# Autodesk Inventor assembly: Baugruppe1
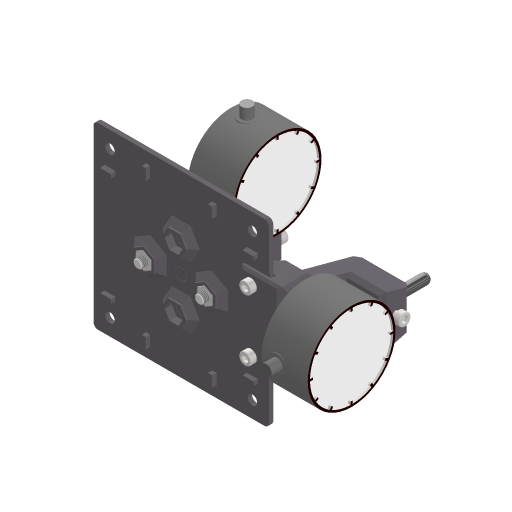
[picture p0: Inventor's stored thumbnail of the model, 512x512]
Saved by Autodesk Inventor 2023.2 (Build 272271000, 271)
## iProperties
Created: 2024-12-10
Part Number: Baugruppe1
Document SubType Name: Assembly
Designer: Nils Bade
Author: Nils Bade
## Documents named in this file (11)
- C:\Users\nilsb\Documents\Inventor\Projektarbeit-Bade\RatRig_modified\ProbeHead\ProbeAntennas\Vermessungsbauteile\MessuhrHalterAssembly.iam
- MessuhrHalterAssembly.iam
- C:\Users\nilsb\Documents\Inventor\Projektarbeit-Bade\RatRig_modified\ProbeHead\ProbeAntennas\Vermessungsbauteile\MessuhrHalter-BasePlate.ipt
- C:\Users\nilsb\Documents\Inventor\Projektarbeit-Bade\RatRig_modified\ProbeHead\ProbeAntennas\Vermessungsbauteile\MessuhrXYKlemme.ipt
- C:\Users\nilsb\Documents\Inventor\Projektarbeit-Bade\RatRig_modified\ProbeHead\ProbeAntennas\Vermessungsbauteile\MessuhrZKlemme.ipt
- C:\Users\nilsb\Documents\Inventor\Projektarbeit-Bade\RatRig_modified\ProbeHead\ProbeAntennas\Vermessungsbauteile\Messuhr-Dummy.ipt
- C:\Users\nilsb\Documents\Inventor\Projektarbeit-Bade\Schrauben\Cap Head Screw M3x12 v2.ipt
- C:\Users\nilsb\Documents\Inventor\Projektarbeit-Bade\Schrauben\Cap Head Screw M3x8 v2.ipt
- C:\Users\nilsb\Documents\Inventor\Projektarbeit-Bade\RatRig_Standards\Hex Nut - M3 v2.ipt
- C:\Users\nilsb\Documents\Inventor\Projektarbeit-Bade\RatRig_Standards\Hex Nut - M4 DIN934.ipt
- C:\Users\nilsb\Documents\Inventor\Projektarbeit-Bade\Schrauben\Cap Head Screw M4x10 - DIN912.ipt
## Components (18 placed, 9 different names)
1. MessuhrHalter-BasePlate:1 — Passend:1, Passend:2, Passend:3, Passend:4, Passend:5, Passend:6, Passend:27, Passend:28, Winkel:5, Winkel:6, Passend:29, Passend:30
2. MessuhrXYKlemme:1 — Passend:1, Passend:2, Passend:6, Tangential:2, Passend:8, Passend:10, Passend:11, Passend:12, Passend:13, Winkel:1, Winkel:2, Passend:17, Passend:18, Passend:31, Passend:32, Passend:33, Passend:34
3. MessuhrZKlemme:1 — Passend:3, Passend:4, Passend:5, Passend:7, Tangential:1, Passend:9, Passend:14, Passend:19, Passend:20, Passend:21, Passend:22, Winkel:3, Winkel:4, Passend:25, Passend:26
4. Messuhr-Dummy:1 — Tangential:2, Passend:8
5. Messuhr-Dummy:2 — Passend:7, Tangential:1
6. Cap Head Screw M3x12 v2:1 — Passend:11, Passend:12, Passend:16
7. Cap Head Screw M3x12 v2:2 — Passend:10, Passend:13, Passend:15
8. Cap Head Screw M3x8 v2:1 — Passend:9, Passend:14
9. Hex Nut - M3 v2:1 — Passend:16, Winkel:2, Passend:17
10. Hex Nut - M3 v2:2 — Passend:15, Winkel:1, Passend:18
11. Hex Nut - M3 v2:3 — Passend:23, Winkel:3, Passend:25
12. Hex Nut - M3 v2:4 — Passend:24, Winkel:4, Passend:26
13. Cap Head Screw M3x12 v2:3 — Passend:19, Passend:22, Passend:23
14. Cap Head Screw M3x12 v2:4 — Passend:20, Passend:21, Passend:24
15. Hex Nut - M4 DIN934:1 — Passend:28, Winkel:6, Passend:30
16. Hex Nut - M4 DIN934:2 — Passend:27, Winkel:5, Passend:29
17. Cap Head Screw M4x10 - DIN912:1 — Passend:31, Passend:34
18. Cap Head Screw M4x10 - DIN912:2 — Passend:32, Passend:33
## Relationships (42: Mate 34, Angle 6, Tangent 2)
- Passend:1 [Mate]: MessuhrHalter-BasePlate:1 ↔ MessuhrXYKlemme:1
- Passend:2 [Mate]: MessuhrHalter-BasePlate:1 ↔ MessuhrXYKlemme:1
- Passend:3 [Mate]: MessuhrHalter-BasePlate:1 ↔ MessuhrZKlemme:1
- Passend:4 [Mate]: MessuhrHalter-BasePlate:1 ↔ MessuhrZKlemme:1
- Passend:5 [Mate]: MessuhrHalter-BasePlate:1 ↔ MessuhrZKlemme:1
- Passend:6 [Mate]: MessuhrHalter-BasePlate:1 ↔ MessuhrXYKlemme:1
- Passend:7 [Mate]: MessuhrZKlemme:1 ↔ Messuhr-Dummy:2
- Tangential:1: MessuhrZKlemme:1 ↔ Messuhr-Dummy:2
- Tangential:2: MessuhrXYKlemme:1 ↔ Messuhr-Dummy:1
- Passend:8 [Mate]: MessuhrXYKlemme:1 ↔ Messuhr-Dummy:1
- Passend:9 [Mate]: MessuhrZKlemme:1 ↔ Cap Head Screw M3x8 v2:1
- Passend:10 [Mate]: MessuhrXYKlemme:1 ↔ Cap Head Screw M3x12 v2:2
- Passend:11 [Mate]: MessuhrXYKlemme:1 ↔ Cap Head Screw M3x12 v2:1
- Passend:12 [Mate]: MessuhrXYKlemme:1 ↔ Cap Head Screw M3x12 v2:1
- Passend:13 [Mate]: MessuhrXYKlemme:1 ↔ Cap Head Screw M3x12 v2:2
- Passend:14 [Mate] (0.75 mm): MessuhrZKlemme:1 ↔ Cap Head Screw M3x8 v2:1
- Passend:15 [Mate]: Cap Head Screw M3x12 v2:2 ↔ Hex Nut - M3 v2:2
- Passend:16 [Mate]: Cap Head Screw M3x12 v2:1 ↔ Hex Nut - M3 v2:1
- Winkel:1 [Angle] (0 deg): MessuhrXYKlemme:1 ↔ Hex Nut - M3 v2:2
- Winkel:2 [Angle] (0 deg): MessuhrXYKlemme:1 ↔ Hex Nut - M3 v2:1
- Passend:17 [Mate]: MessuhrXYKlemme:1 ↔ Hex Nut - M3 v2:1
- Passend:18 [Mate]: MessuhrXYKlemme:1 ↔ Hex Nut - M3 v2:2
- Passend:19 [Mate]: MessuhrZKlemme:1 ↔ Cap Head Screw M3x12 v2:3
- Passend:20 [Mate]: MessuhrZKlemme:1 ↔ Cap Head Screw M3x12 v2:4
- Passend:21 [Mate]: MessuhrZKlemme:1 ↔ Cap Head Screw M3x12 v2:4
- Passend:22 [Mate]: MessuhrZKlemme:1 ↔ Cap Head Screw M3x12 v2:3
- Passend:23 [Mate]: Hex Nut - M3 v2:3 ↔ Cap Head Screw M3x12 v2:3
- Passend:24 [Mate]: Hex Nut - M3 v2:4 ↔ Cap Head Screw M3x12 v2:4
- Winkel:3 [Angle] (0 deg): MessuhrZKlemme:1 ↔ Hex Nut - M3 v2:3
- Winkel:4 [Angle] (0 deg): MessuhrZKlemme:1 ↔ Hex Nut - M3 v2:4
- Passend:25 [Mate]: MessuhrZKlemme:1 ↔ Hex Nut - M3 v2:3
- Passend:26 [Mate]: MessuhrZKlemme:1 ↔ Hex Nut - M3 v2:4
- Passend:27 [Mate]: MessuhrHalter-BasePlate:1 ↔ Hex Nut - M4 DIN934:2
- Passend:28 [Mate]: MessuhrHalter-BasePlate:1 ↔ Hex Nut - M4 DIN934:1
- Winkel:5 [Angle] (0 deg): MessuhrHalter-BasePlate:1 ↔ Hex Nut - M4 DIN934:2
- Winkel:6 [Angle] (0 deg): MessuhrHalter-BasePlate:1 ↔ Hex Nut - M4 DIN934:1
- Passend:29 [Mate]: MessuhrHalter-BasePlate:1 ↔ Hex Nut - M4 DIN934:2
- Passend:30 [Mate]: MessuhrHalter-BasePlate:1 ↔ Hex Nut - M4 DIN934:1
- Passend:31 [Mate]: MessuhrXYKlemme:1 ↔ Cap Head Screw M4x10 - DIN912:1
- Passend:32 [Mate]: MessuhrXYKlemme:1 ↔ Cap Head Screw M4x10 - DIN912:2
- Passend:33 [Mate]: MessuhrXYKlemme:1 ↔ Cap Head Screw M4x10 - DIN912:2
- Passend:34 [Mate]: MessuhrXYKlemme:1 ↔ Cap Head Screw M4x10 - DIN912:1
